# Autodesk Inventor assembly: 045-DP(F,D-166-3)
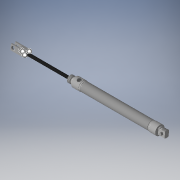
[picture p0: Inventor's stored thumbnail of the model, 180x180]
Saved by Autodesk Inventor 2017 (Build 210142000, 142)
## iProperties
Category: PARTsolutions
Company: BIMBA
Created: 2016-11-05
Part Number: 045-DP(F,D-166-3)
Catalog Web Link: www.cadenas.de
Description: Original Line Standard Air Cylinders-
Vendor: BIMBA
Document SubType Name: Assembly
Designer: psAdmin
Manufacturer: BIMBA
Mass: 24.8714 g
Surface Area: 284.573 cm^2
Volume: 24.8714 cm^3
Density: 1 g/cm^3
PSOL_IDENT_0: {$CADENAS_DATA\23d-libs\bimba\bimba\bimba_imperial\bimba_full_line\original_line_cylinders\standard_
PSOL_IDENT_1: air_cylinders\standard_air_cylinder_asmtab.prj},323 {VTYP=3D},{STYP=ASSTAB},{NB=045-DP(F,D-166-3)},{
PSOL_IDENT_2: LINA=045-DP},{NN=Original Line Standard Air Cylinders},{DATE=22.09.2016 13:52:24},{GEOMDATE=11.07.20
PSOL_IDENT_3: 16 10:37:18},{VERSION=},{LINEID=50},{LINESUBID=-1},{WBVAR=STROKE,ACTING,MNT,DER,NR,BM,CO,OO,VO,M,EE,
PSOL_IDENT_4: EEL,K,Q,Y,G,T,B,H,SER,SR,NT,W,HL,STPT1,STPT2,STPT3,STPT4,MB,PB,PRC,TB,MN}  {NB=045-DP(F,D-166-3)},{L
PSOL_IDENT_5: INA=045-DP},{KT=DUMMY},{PN=045-DP},{PNC=045-DP(F,D-166-3)},{PNA=(D-166-3)},{DASH=-},{BORE1=0.7500000
PSOL_IDENT_6: 0},{BORE=3/4\" (04)},{BOREPN=04},{STROKE=5.000},{STROKEALG=[0.011:50/0.001]},{STROKE1=5.000},{ACTING=
PSOL_IDENT_7: D},{ACTINGALG= '' , 'Single Acting (SA)' , 'R' , 'Reverse Single Acting (SA)' , 'D' , 'Double Acting
PSOL_IDENT_8: (SA)' },{ACTINGPN=D},{MNT=P},{MNTALG= '' , 'Front Nose Mounting (SA)' , 'P' , 'Rear Pivot Mounting
PSOL_IDENT_9: (SA)' , 'XP' , 'Double End or Pivot Mounting (SA)' , 'X' , 'Double End Mounting (SA)' , 'BF' , 'Fron
PSOL_IDENT_10: t Block Mounting (SA)' , 'BR' , 'Rear Block Mounting for Vertical Positioning (SA)' , 'BFT' , 'Front
PSOL_IDENT_11: Block Trunnion Mounting (SA)' , 'BRT' , 'Rear Block Trunnion Mounting (SA)' },{TYPE=},{MNTPN=P},{DE
PSOL_IDENT_12: R=},{DERALG= '' , 'N/A' },{NR=},{NRALG= '' , 'N/A' },{NRPN=},{BM=},{BMALG= '' , 'N/A' },{BMPN=},{CO=
PSOL_IDENT_13: },{COALG= '' , 'N/A' },{OO=},{OOALG= '', 'N/A' },{OOPN=},{VO=Z},{VOALG= 'Z' , 'N/A' },{VOPN=},{OOVOP
PSOL_IDENT_14: N=},{M=},{MALG= '', 'Without Magnet', 'M', 'With Magnet' },{EE=},{EEL=0.000},{EEMAX=45.0000},{EEALG=
PSOL_IDENT_15: '', 'Without Extra Extension', 'EE', 'With Extra Extension' },{EELALG=0},{EEPN=},{EEPN1=0.000},{K=}
PSOL_IDENT_16: ,{KALG= '', 'Standard' , 'K' , 'Ports Rotated 90deg K' },{KPN=},{Q=},{QALG= '' , 'N/A' },{QPN=},{Y=}
PSOL_IDENT_17: ,{YALG= '' , 'Without Pivot Bushing' , 'Y' , 'With Pivot Bushing' },{YPN=},{YCON=},{F=},{FALG= '', '
PSOL_IDENT_18: Non-Coated (Standard)', 'F', 'Molycoated' },{FPN=},{G=},{GPN=},{GPN99=},{T=},{TALG= '' , 'Standard -
PSOL_IDENT_19: 20° to 200°F (-29° to 95°C)' , 'N' , 'Low Temperature' , 'V' , 'High Temperature' },{NPN=},{VPN=},{B=
PSOL_IDENT_20: },{BALG= '', 'W/out Bumpers' , 'B' , 'W/ Bumpers' },{BPN=},{H=},{HALG= '', 'N/A' },{HPN=},{SER=},{SE
PSOL_IDENT_21: RALG= '' , 'Without Spring Extend/Return' , 'JS' , 'With Spring Return' , 'JR' , 'With Spring Extend'
PSOL_IDENT_22: },{SR=C},{SRALG= 'C' , 'Standard Blackened Carbon Steel' , 'SR' , 'Stainless Steel [SR]' },{SRPN=},
PSOL_IDENT_23: {SRCON=1},{NT=},{NTPN=},{W=},{WALG= '' , 'Without Wiper' , 'W' , 'With Wiper' },{WPN=},{E=},{EALG= ''
PSOL_IDENT_24: , 'Standard Seals/Lube' , 'E' , 'Non-Lube Seals/Lube' },{EPN=},{HL=},{HLALG= '' , 'Without Low Pres
PSOL_IDENT_25: sure Hydraulic' , 'HL' , 'With Low Pressure Hydraulic' },{ST=},{STALG= '' , 'N/A' },{STPT1=},{STPT1A
PSOL_IDENT_26: LG= '' , 'N/A' },{STPT2=},{STPT2ALG= '' , 'N/A' },{STPT3=},{STPT3ALG= '' , 'N/A' },{STPT4=},{STPT4AL
PSOL_IDENT_27: G= '' , 'N/A' },{STPN=},{MB=},{MBALG= '' , 'N/A' },{MBPN=},{MBPNALL=},{MBPNALLREAR=},{PB=},{PBALG= ''
PSOL_IDENT_28: , 'Without Pivot Bracket' , 'D-167' , 'D-167' },{PBPN=},{PBPNALL=D-167},{PRC=F,D-166-3},{PRCALG= ''
PSOL_IDENT_29: , 'W/out Pivot Rod Clevis' , 'F,D-166-3' , 'D-166-3 (front)' },{PRCPN=(F,D-166-3)},{PRCPNALL=D-166-
PSOL_IDENT_30: 3},{TB=},{TBALG= '' , 'N/A' },{TBPN=},{TBPNALL=},{MN=},{MNALG= '' , 'Without Mounting Nut' , 'F,D-9'
PSOL_IDENT_31: , 'D-9 (front)' , 'R,D-9' , 'D-9 (rear)', '2x,D-9' , 'D-9 (front & rear)' },{MNPN=},{MNCONF=},{MNCO
PSOL_IDENT_32: NR=},{TLEN=6.2555},{FRAC=32.7500},{RGCON=},{RGDACCON=R},{RHCON=P},{RHCON1=P},{RHCONON=1},{RHACCON=},
PSOL_IDENT_33: {FNUTCON=0},{RNUTCON=0},{FNUTPN=D-9},{RNUTPN=D-9},{FNUTTRANS=0.0000},{RNUTTRANS=0.0000},{VHOLECON=0}
PSOL_IDENT_34: ,{A1=1.5940},{A1N=0.8750},{A1P=1.5940},{A1B=1.5940},{A4=0.2525},{A4N=0.3130},{A4P=0.2525},{A5=0.0300
PSOL_IDENT_35: },{A1H=1.594},{A1NH=0.5310},{A1PH=1.5940},{A1BH=1.0940},{A1SH=1.2190},{A2H=0.2190},{A2NH=0.2190},{LE
PSOL_IDENT_36: NGTH=3.7500},{LENGTH1=3.7500},{LENGTH2=3.8100},{MUL=5.0000},{MUL11=5.0000},{MUL22=13.45},{MUL33=8.45
PSOL_IDENT_37: 00},{MUL2=5.0000},{MUL211=5.0000},{MUL222=2.6900},{MUL233=1.6900},{SSS=10.0000},{RGLEN=1.3715},{RHLE
PSOL_IDENT_38: N=1.1230},{SSS1=6.0000},{A13=1.3120},{DIF=0.0000},{G5=0.6250},{ON=0},{SSADD=0.0000},{BADD=0.0000},{M
PSOL_IDENT_39: ADD=0.0000},{NVADD=0.0000},{TRACKL=5.9655},{TRACKCON=D-74168},{TRIMCON=0},{TRIMCON1=0},{PINCON=D-51}
PSOL_IDENT_40: ,{FSPACE=0.6091},{SPACE=0.0964},{TEXT=0.1688},{S1=1.0000},{D1=0.8325},{D1N=0.8050},{D1B=0.8625},{D1P=
PSOL_IDENT_41: 0.8325},{FA=0.940},{RA=0.9400},{PPATH=standard_air_cylinder_asmtpl.prj},{MATALGHTML=<b>Standard Orig
PSOL_IDENT_42: inal Line:</b><dl><dt>Rod:</dt><dd>- Stainless Steel</dd><dd>&nbsp;&nbsp;(5/16 9/16 Bores)</dd><dd>-
PSOL_IDENT_43: High Strength Carbon Steel</dd><dd>&nbsp;&nbsp;(3/4 3 Bore)</dd><dd>- Stainless Steel</dd><dd>&nbsp
PSOL_IDENT_44: ;&nbsp;(X style DXP/DX/DXDE)</dd><dt>Bearings:</dt><dd>- Sintered Bronze</dd><dt>Body:</dt><dd>- 304
PSOL_IDENT_45: Stainless Steel</dd><dt>End Caps:</dt><dd>- Aluminum</dd><dt>Seals:</dt><dd>- Buna N</dd></dl>},{AS
PSOL_IDENT_46: SCFGPRA=04DP},{MBPNA=},{MNPNA=},{PRCPNA=(D-166-3)},{ASSOPTACC=STPT4},{A=8.75},{HADD=0.0000},{WFL=0.2
PSOL_IDENT_47: 5},{QADD=0.000},{QADD1=0.440},{TEST=5.0000},{MNTB=},{STDNUTF=0},{STDNUTR=0},{STRK2D=0},{X2D=2},{STRO
PSOL_IDENT_48: KESW=5.000},{EESW=0.000},{FCD=0},{BCD=0},{RCD=0},{CUSTADD=4.000},{FT=1/4-28 UNF-2A},{FT1=1/4-28 UNF-
PSOL_IDENT_49: 2A},{FT2=5/8-18 UNF-2A},{PORT=1/8 NPT},{FT11=1/2-20 UNF-2A},{FT12=5/8-18 UNF-2A}
NN: Original Line Standard Air Cylinders
NT: Standard Male Thread
NB: 045-DP(F,D-166-3)
NBSYN: $PNC.
LINA: 045-DP
PN: 045-DP
PNA: (D-166-3)
BORE: 3/4" [04]
STROKE: 5.000
ACTING: Double [D]
MNT: Rear Pivot [P]
DER: N/A
NR: N/A
BM: N/A
CO: N/A
OO: N/A
VO: N/A
M: Without Magnet Piston
EE: Standard Rod Extension
EEL: 0.000
K: Standard
Q: N/A
Y: Standard Pivot Style
G: Standard Grease Lube
T: Standard -20° to 200°F (-29° to 95°C)
B: Without Bumpers
H: N/A
SER: Without Failsafe Spring Extend/Return
SR: Standard Blackened Carbon Steel
W: Without Wiper
HL: Standard 250 PSI Air
STPT1: N/A
STPT2: N/A
STPT3: N/A
STPT4: N/A
MB: N/A
PB: Without Pivot Bracket
PRC: D-166-3 (front)
TB: N/A
MN: Without Mounting Nut
A: 8.75
SUPPLIER: BIMBA
ARTICLENO: 045-DP(F,D-166-3)
BOMINFO: 045-DP
CREATOR: CADENAS GmbH
Title: 045-DP
Author: Cadenas PARTsolutions
## Documents named in this file (6)
- \\Mac\Home\Desktop\bunnybots 2016\15102898-16-Bunnybot-CAD\Bunnybot-To_be_renamed\15102898-16-A-0000\15102898-16-A-0900\Imported Components\AIS2015\045-DP(F,D-166-3).iam
- \\Mac\Home\Desktop\bunnybots 2016\15102898-16-Bunnybot-CAD\Bunnybot-To_be_renamed\15102898-16-A-0000\15102898-16-A-0900\Imported Components\AIS2015\045-DPC(F,D-166-3)0000_0_dummy.ipt
- \\Mac\Home\Desktop\bunnybots 2016\15102898-16-Bunnybot-CAD\Bunnybot-To_be_renamed\15102898-16-A-0000\15102898-16-A-0900\Imported Components\AIS2015\04R000-0_rod_guide.ipt
- \\Mac\Home\Desktop\bunnybots 2016\15102898-16-Bunnybot-CAD\Bunnybot-To_be_renamed\15102898-16-A-0000\15102898-16-A-0900\Imported Components\AIS2015\04R-6_25550C.ipt
- \\Mac\Home\Desktop\bunnybots 2016\15102898-16-Bunnybot-CAD\Bunnybot-To_be_renamed\15102898-16-A-0000\15102898-16-A-0900\Imported Components\AIS2015\04P0000_rear_head.ipt
- \\Mac\Home\Desktop\bunnybots 2016\15102898-16-Bunnybot-CAD\Bunnybot-To_be_renamed\15102898-16-A-0000\15102898-16-A-0900\Imported Components\AIS2015\D-166-3-dummy.ipt
## Components (5 placed, 5 different names)
1. 045-DPC(F,D-166-3)0000_0_dummy:1
2. 04R000-0_rod_guide:1 — Mate:5, Mate:6
3. 04R-6_25550C:1 — Mate:5, Mate:6, Mate:7, Mate:8
4. 04P0000_rear_head:1 — Mate:7, Mate:8
5. D-166-3-dummy:1
## Relationships (4: Mate 4)
- Mate:5: 04R000-0_rod_guide:1 ↔ 04R-6_25550C:1
- Mate:6: 04R000-0_rod_guide:1 ↔ 04R-6_25550C:1
- Mate:7: 04R-6_25550C:1 ↔ 04P0000_rear_head:1
- Mate:8: 04R-6_25550C:1 ↔ 04P0000_rear_head:1
